# Autodesk Inventor assembly: topBottom
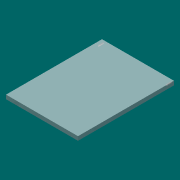
[picture p0: Inventor's stored thumbnail of the model, 180x180]
Saved by Autodesk Inventor 2016 (Build 200138000, 138)
## iProperties
Created: 2015-10-19
Part Number: topBottom
Document SubType Name: Assembly
Designer: Sawaiz
Author: Sawaiz
## Documents named in this file (3)
- C:\Users\Sawaiz\OneDrive\projects\modularRICH\frame\topBottom.iam
- C:\Users\Sawaiz\OneDrive\projects\modularRICH\frame\topBottom.ipt
- C:\Users\Sawaiz\OneDrive\projects\modularRICH\modularRICH.xlsx
## Components (1 placed, 1 different names)
1. topBottom:1
## Named parameters: acrylicThickness = 6.35 mm, aerogelThickness = 30 mm, height = 101.6 mm, width = 101.6 mm, depth = 152.4 mm, mirrorAngle = 5 deg, detectorWidth = 52 mm, detectorHeight = 52 mm, mirrorThickness = 3.175 mm, fresnelThickness = 0.1 mm, grooveDensity = 100, focalLength = 76.2 mm, ior = 1.49, centerThickness = 1.524 mm, fresnelAngle = 90 deg, fresnelEffectiveDiameter = 76.2 mm, mirrorSuppourtWidth = 38.1 mm, backGrooveBit = 4.8006 mm, sensorHolderWidth = 88.9 mm, sensorHolderHeight = 88.9 mm, sensorHolderSensorHeight = 53.975 mm, sensorHolderSensorWidth = 53.975 mm, oRingWidth = 3.175 mm, sensorHolderORingID = 203.2 mm, sensorHolderFlushORingID = 304.8 mm, frontBackORingID = 419.1 mm, mirrorGroove = 19.05 mm, backMirrorGroove = 6.35 mm, compressionPercent = 40, mirrorGrooveFillet = 6.35 mm, fresnelChamfer = 6.35 mm, mirrorGrooveDrill = 6.35 mm, mirrorGrooveMill = 3.175 mm, fresnelMirrorChamfer = 6.35 mm, detectorOpeningHeight = 76.2 mm, detectorOpeningWidth = 76.2 mm
